# Autodesk Inventor assembly: SPM_assembly_V2
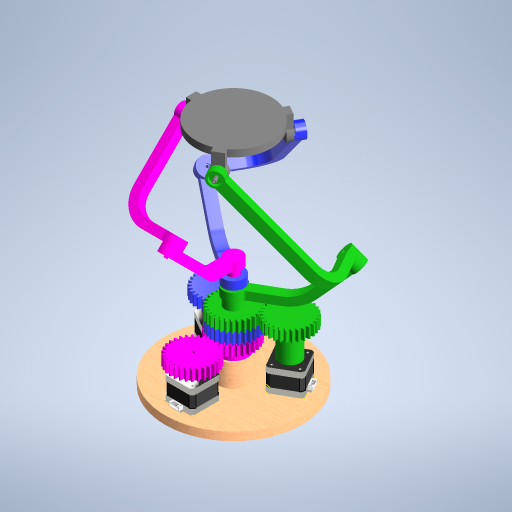
[picture p0: Inventor's stored thumbnail of the model, 512x512]
Saved by Autodesk Inventor 2024 (Build 280153000, 153)
## iProperties
Created: 2023-10-30
Part Number: SPM_assembly_V2
Document SubType Name: Assembly
Designer: MATEO
Author: MATEO
## Documents named in this file (17)
- C:\Users\MATEO\Desktop\PROYECTO DE GRADO-IMEC\3-RRR_SPM_CAD\3-RRR_SPM_CAD_V2\SPM_assembly_V2.iam
- C:\Users\MATEO\Desktop\PROYECTO DE GRADO-IMEC\3-RRR_SPM_CAD\3-RRR_SPM_CAD_V2\fixed_base.ipt
- C:\Users\MATEO\Desktop\PROYECTO DE GRADO-IMEC\3-RRR_SPM_CAD\3-RRR_SPM_CAD_V2\NEMA_17.ipt
- C:\Users\MATEO\Desktop\PROYECTO DE GRADO-IMEC\3-RRR_SPM_CAD\3-RRR_SPM_CAD_V2\link_gear_3.ipt
- C:\Users\MATEO\Desktop\PROYECTO DE GRADO-IMEC\3-RRR_SPM_CAD\3-RRR_SPM_CAD_V2\input_gear_3.ipt
- C:\Users\MATEO\Desktop\PROYECTO DE GRADO-IMEC\3-RRR_SPM_CAD\3-RRR_SPM_CAD_V2\link_gear_2.ipt
- C:\Users\MATEO\Desktop\PROYECTO DE GRADO-IMEC\3-RRR_SPM_CAD\3-RRR_SPM_CAD_V2\input_gear_2.ipt
- C:\Users\MATEO\Desktop\PROYECTO DE GRADO-IMEC\3-RRR_SPM_CAD\3-RRR_SPM_CAD_V2\link_gear_1.ipt
- C:\Users\MATEO\Desktop\PROYECTO DE GRADO-IMEC\3-RRR_SPM_CAD\3-RRR_SPM_CAD_V2\input_gear_1.ipt
- C:\Users\MATEO\Desktop\PROYECTO DE GRADO-IMEC\3-RRR_SPM_CAD\3-RRR_SPM_CAD_V2\proximal_link_1.ipt
- C:\Users\MATEO\Desktop\PROYECTO DE GRADO-IMEC\3-RRR_SPM_CAD\3-RRR_SPM_CAD_V2\proximal_link_2.ipt
- C:\Users\MATEO\Desktop\PROYECTO DE GRADO-IMEC\3-RRR_SPM_CAD\3-RRR_SPM_CAD_V2\proximal_link_3.ipt
- C:\Users\MATEO\Desktop\PROYECTO DE GRADO-IMEC\3-RRR_SPM_CAD\3-RRR_SPM_CAD_V2\distal_link_1.ipt
- C:\Users\MATEO\Desktop\PROYECTO DE GRADO-IMEC\3-RRR_SPM_CAD\3-RRR_SPM_CAD_V2\distal_link_2.ipt
- C:\Users\MATEO\Desktop\PROYECTO DE GRADO-IMEC\3-RRR_SPM_CAD\3-RRR_SPM_CAD_V2\distal_link_3.ipt
- C:\Users\MATEO\Desktop\PROYECTO DE GRADO-IMEC\3-RRR_SPM_CAD\3-RRR_SPM_CAD_V2\mobile_platform.ipt
- C:\Users\MATEO\Desktop\PROYECTO DE GRADO-IMEC\3-RRR_SPM_CAD\3-RRR_SPM_CAD_V2\encoder_cover.ipt
## Components (20 placed, 16 different names)
1. fixed_base:1 — Flush:1, Flush:2, Flush:3, Insert:2, Mate:15, Insert:17
2. link_gear_3:1 — Insert:2, Rotation:1, Insert:4, Insert:10, Mate:6
3. input_gear_3:1 — Insert:3, Rotation:1
4. link_gear_2:1 — Insert:4, Rotation:2, Insert:6, Insert:9, Mate:5
5. input_gear_2:1 — Insert:5, Rotation:2
6. link_gear_1:1 — Insert:6, Rotation:3, Insert:8, Mate:4
7. input_gear_1:1 — Insert:7, Rotation:3
8. proximal_link_1:1 — Insert:8, Mate:4, Angle:1, Insert:11
9. proximal_link_2:1 — Insert:9, Mate:5, Angle:2, Insert:12
10. proximal_link_3:1 — Insert:10, Mate:6, Angle:3, Insert:13
11. distal_link_1:1 — Insert:11, Insert:14, Mate:19
12. distal_link_2:1 — Insert:12, Mate:8, Mate:18
13. distal_link_3:1 — Insert:13, Mate:7, Mate:17
14. mobile_platform:1 — Insert:14, Mate:7, Mate:8, Flush:4, Mate:10, Flush:5, Mate:12, Flush:6, Mate:14
15. NEMA_17:1 — Insert:3, Angle:3, Mate:15, Insert:16, Mate:16
16. encoder_cover:1 — Insert:16, Mate:16, Insert:17
17. NEMA_17:2 — Insert:5, Angle:2
18. encoder_cover:2
19. NEMA_17:3 — Insert:7, Angle:1
20. encoder_cover:3
## Component patterns: (3 elements, first: NEMA_17:1 + encoder_cover:1)
## Relationships (43: Mate 16, Insert 15, Flush 6, RelateRotation 3, Angle 3)
- Flush:1: fixed_base:1
- Flush:2: fixed_base:1
- Flush:3: fixed_base:1
- Insert:2: fixed_base:1 ↔ link_gear_3:1
- Insert:3: input_gear_3:1 ↔ NEMA_17:1
- Rotation:1 [RelateRotation] (1 ul): link_gear_3:1 ↔ input_gear_3:1
- Insert:4: link_gear_3:1 ↔ link_gear_2:1
- Insert:5: input_gear_2:1 ↔ NEMA_17:2
- Rotation:2 [RelateRotation] (1 ul): link_gear_2:1 ↔ input_gear_2:1
- Insert:6: link_gear_2:1 ↔ link_gear_1:1
- Insert:7: input_gear_1:1 ↔ NEMA_17:3
- Rotation:3 [RelateRotation] (1 ul): link_gear_1:1 ↔ input_gear_1:1
- Insert:8: link_gear_1:1 ↔ proximal_link_1:1
- Mate:4: link_gear_1:1 ↔ proximal_link_1:1
- Insert:9: link_gear_2:1 ↔ proximal_link_2:1
- Mate:5: link_gear_2:1 ↔ proximal_link_2:1
- Insert:10: link_gear_3:1 ↔ proximal_link_3:1
- Mate:6: link_gear_3:1 ↔ proximal_link_3:1
- Angle:1 (180 deg): proximal_link_1:1 ↔ NEMA_17:3
- Angle:2 (180 deg): proximal_link_2:1 ↔ NEMA_17:2
- Angle:3 (180 deg): proximal_link_3:1 ↔ NEMA_17:1
- Insert:11: proximal_link_1:1 ↔ distal_link_1:1
- Insert:12: proximal_link_2:1 ↔ distal_link_2:1
- Insert:13: proximal_link_3:1 ↔ distal_link_3:1
- Insert:14: distal_link_1:1 ↔ mobile_platform:1
- Mate:7: distal_link_3:1 ↔ mobile_platform:1
- Mate:8: distal_link_2:1 ↔ mobile_platform:1
- Flush:4 (53 mm): mobile_platform:1
- Mate:9
- Mate:10: mobile_platform:1
- Flush:5 (53 mm): mobile_platform:1
- Mate:11
- Mate:12: mobile_platform:1
- Flush:6 (53 mm): mobile_platform:1
- Mate:13
- Mate:14: mobile_platform:1
- Mate:15: fixed_base:1 ↔ NEMA_17:1
- Insert:16: NEMA_17:1 ↔ encoder_cover:1
- Mate:16: NEMA_17:1 ↔ encoder_cover:1
- Insert:17: fixed_base:1 ↔ encoder_cover:1
- Mate:17: distal_link_3:1
- Mate:18: distal_link_2:1
- Mate:19: distal_link_1:1
